# Autodesk Inventor assembly: Pulley_GT2_5mm pitch_240-tooth
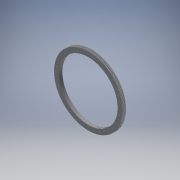
[picture p0: Inventor's stored thumbnail of the model, 180x180]
Saved by Autodesk Inventor 2018.3 (Build 223284000, 284)
## iProperties
Created: 2020-01-26
Part Number: Pulley_GT2_5mm pitch_240-tooth
Document SubType Name: Assembly
Designer: dillmcke
Author: dillmcke
## Documents named in this file (2)
- C:\Users\dillmcke\Documents\GrabCAD\Infinite Recharge 2020\Build season\Pulley_GT2_5mm pitch_240-tooth.iam
- C:\Users\dillmcke\Documents\GrabCAD\Infinite Recharge 2020\Build season\Pulley_GT2_5mm pitch_240-tooth.ipt
## Components (12 placed, 1 different names)
1. Pulley_GT2_5mm pitch_240-tooth:1 — Flush:1, Mate:1, Mate:2, Mate:5, Mate:6, Mate:13, Mate:14, Mate:15, Mate:24
2. Pulley_GT2_5mm pitch_240-tooth:2 — Flush:1, Flush:2, Mate:1, Mate:2, Mate:3, Mate:4
3. Pulley_GT2_5mm pitch_240-tooth:3 — Flush:2, Flush:3, Mate:3, Mate:4
4. Pulley_GT2_5mm pitch_240-tooth:4 — Flush:3, Mate:5, Mate:6, Mate:23
5. Pulley_GT2_5mm pitch_240-tooth:5 — Mate:11, Mate:12, Flush:6, Mate:25
6. Pulley_GT2_5mm pitch_240-tooth:6 — Mate:7, Mate:8, Flush:4
7. Pulley_GT2_5mm pitch_240-tooth:7 — Flush:5, Mate:9, Mate:10, Mate:11, Mate:12, Flush:6, Mate:13, Mate:14, Mate:15
8. Pulley_GT2_5mm pitch_240-tooth:8 — Mate:7, Mate:8, Flush:4, Flush:5, Mate:9, Mate:10
9. Pulley_GT2_5mm pitch_240-tooth:9 — Mate:16, Mate:17, Flush:7
10. Pulley_GT2_5mm pitch_240-tooth:10 — Mate:16, Mate:17, Flush:7, Mate:18, Flush:8, Mate:19, Mate:23
11. Pulley_GT2_5mm pitch_240-tooth:11 — Mate:18, Flush:8, Mate:19, Mate:20, Flush:9, Mate:21, Mate:24
12. Pulley_GT2_5mm pitch_240-tooth:12 — Mate:20, Flush:9, Mate:21, Mate:25
## Relationships (33: Mate 24, Flush 9)
- Flush:1: Pulley_GT2_5mm pitch_240-tooth:1 ↔ Pulley_GT2_5mm pitch_240-tooth:2
- Flush:2: Pulley_GT2_5mm pitch_240-tooth:2 ↔ Pulley_GT2_5mm pitch_240-tooth:3
- Flush:3: Pulley_GT2_5mm pitch_240-tooth:3 ↔ Pulley_GT2_5mm pitch_240-tooth:4
- Mate:1: Pulley_GT2_5mm pitch_240-tooth:1 ↔ Pulley_GT2_5mm pitch_240-tooth:2
- Mate:2: Pulley_GT2_5mm pitch_240-tooth:1 ↔ Pulley_GT2_5mm pitch_240-tooth:2
- Mate:3: Pulley_GT2_5mm pitch_240-tooth:2 ↔ Pulley_GT2_5mm pitch_240-tooth:3
- Mate:4: Pulley_GT2_5mm pitch_240-tooth:2 ↔ Pulley_GT2_5mm pitch_240-tooth:3
- Mate:5: Pulley_GT2_5mm pitch_240-tooth:1 ↔ Pulley_GT2_5mm pitch_240-tooth:4
- Mate:6: Pulley_GT2_5mm pitch_240-tooth:1 ↔ Pulley_GT2_5mm pitch_240-tooth:4
- Mate:7: Pulley_GT2_5mm pitch_240-tooth:6 ↔ Pulley_GT2_5mm pitch_240-tooth:8
- Mate:8: Pulley_GT2_5mm pitch_240-tooth:6 ↔ Pulley_GT2_5mm pitch_240-tooth:8
- Flush:4: Pulley_GT2_5mm pitch_240-tooth:6 ↔ Pulley_GT2_5mm pitch_240-tooth:8
- Flush:5: Pulley_GT2_5mm pitch_240-tooth:7 ↔ Pulley_GT2_5mm pitch_240-tooth:8
- Mate:9: Pulley_GT2_5mm pitch_240-tooth:7 ↔ Pulley_GT2_5mm pitch_240-tooth:8
- Mate:10: Pulley_GT2_5mm pitch_240-tooth:7 ↔ Pulley_GT2_5mm pitch_240-tooth:8
- Mate:11: Pulley_GT2_5mm pitch_240-tooth:5 ↔ Pulley_GT2_5mm pitch_240-tooth:7
- Mate:12: Pulley_GT2_5mm pitch_240-tooth:5 ↔ Pulley_GT2_5mm pitch_240-tooth:7
- Flush:6: Pulley_GT2_5mm pitch_240-tooth:5 ↔ Pulley_GT2_5mm pitch_240-tooth:7
- Mate:13: Pulley_GT2_5mm pitch_240-tooth:1 ↔ Pulley_GT2_5mm pitch_240-tooth:7
- Mate:14: Pulley_GT2_5mm pitch_240-tooth:1 ↔ Pulley_GT2_5mm pitch_240-tooth:7
- Mate:15: Pulley_GT2_5mm pitch_240-tooth:1 ↔ Pulley_GT2_5mm pitch_240-tooth:7
- Mate:16: Pulley_GT2_5mm pitch_240-tooth:9 ↔ Pulley_GT2_5mm pitch_240-tooth:10
- Mate:17: Pulley_GT2_5mm pitch_240-tooth:9 ↔ Pulley_GT2_5mm pitch_240-tooth:10
- Flush:7: Pulley_GT2_5mm pitch_240-tooth:9 ↔ Pulley_GT2_5mm pitch_240-tooth:10
- Mate:18: Pulley_GT2_5mm pitch_240-tooth:10 ↔ Pulley_GT2_5mm pitch_240-tooth:11
- Flush:8: Pulley_GT2_5mm pitch_240-tooth:10 ↔ Pulley_GT2_5mm pitch_240-tooth:11
- Mate:19: Pulley_GT2_5mm pitch_240-tooth:10 ↔ Pulley_GT2_5mm pitch_240-tooth:11
- Mate:20: Pulley_GT2_5mm pitch_240-tooth:11 ↔ Pulley_GT2_5mm pitch_240-tooth:12
- Flush:9: Pulley_GT2_5mm pitch_240-tooth:11 ↔ Pulley_GT2_5mm pitch_240-tooth:12
- Mate:21: Pulley_GT2_5mm pitch_240-tooth:11 ↔ Pulley_GT2_5mm pitch_240-tooth:12
- Mate:23: Pulley_GT2_5mm pitch_240-tooth:4 ↔ Pulley_GT2_5mm pitch_240-tooth:10
- Mate:24: Pulley_GT2_5mm pitch_240-tooth:1 ↔ Pulley_GT2_5mm pitch_240-tooth:11
- Mate:25: Pulley_GT2_5mm pitch_240-tooth:5 ↔ Pulley_GT2_5mm pitch_240-tooth:12
